# Autodesk Inventor assembly: base_wall_added
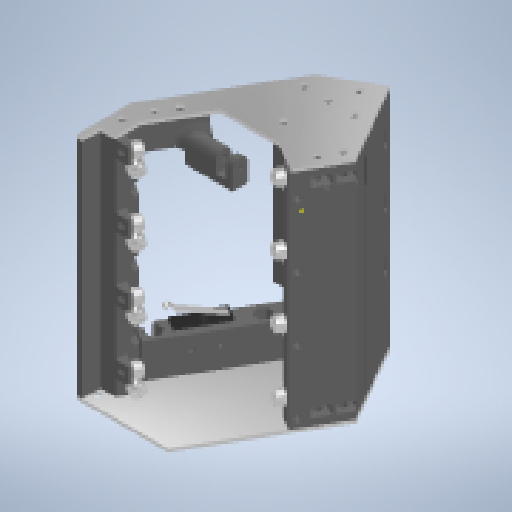
[picture p0: Inventor's stored thumbnail of the model, 512x512]
Saved by Autodesk Inventor 2024.1 (Build 281209000, 209)
## iProperties
Created: 2025-01-18
Part Number: base_wall_added
Document SubType Name: Assembly
Designer: hibik
Author: hibik
## Documents named in this file (4)
- C:\Users\hibik\Documents\Robomech\RESCUE\ORCA\hard\fork\right\base_wall_added.iam
- C:\Users\hibik\Documents\Robomech\RESCUE\ORCA\hard\fork\right\base.iam
- C:\Users\hibik\Documents\Robomech\RESCUE\ORCA\hard\fork\right\base_backwall_setter_upper.ipt
- C:\Users\hibik\Documents\Robomech\RESCUE\ORCA\hard\fork\right\chain_base_connector.ipt
## Components (3 placed, 3 different names)
1. base:1 [sub-assembly] — メイト:1, フラッシュ:1, フラッシュ:2, メイト:2, フラッシュ:3
2. base_backwall_setter_upper:1 — メイト:1, フラッシュ:1, フラッシュ:2
3. chain_base_connector:1 — メイト:2, フラッシュ:3
## Relationships (5: Flush 3, Mate 2)
- メイト:1 [Mate]: base:1 ↔ base_backwall_setter_upper:1
- フラッシュ:1 [Flush]: base:1 ↔ base_backwall_setter_upper:1
- フラッシュ:2 [Flush]: base:1 ↔ base_backwall_setter_upper:1
- メイト:2 [Mate]: base:1 ↔ chain_base_connector:1
- フラッシュ:3 [Flush]: base:1 ↔ chain_base_connector:1
